# Autodesk Inventor assembly: battery gate
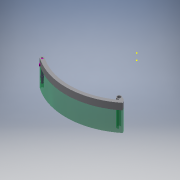
[picture p0: Inventor's stored thumbnail of the model, 180x180]
Saved by Autodesk Inventor 2016 (Build 200138000, 138)
## iProperties
Created: 2015-09-29
Part Number: battery gate
Document SubType Name: Assembly
Designer: Hulbert Office
Author: Hulbert Office
## Documents named in this file (4)
- C:\Users\Hulbert Office\Dropbox\SHF Robotics\battery gate.iam
- C:\Users\Hulbert Office\Dropbox\SHF Robotics\battery gate.ipt
- C:\Users\Hulbert Office\Dropbox\SHF Robotics\battery gate upper.ipt
- C:\Users\Hulbert Office\Dropbox\SHF Robotics\battery gate pin.ipt
## Components (3 placed, 3 different names)
1. battery gate:1 — Mate:1, Mate:2, Mate:3, Mate:4
2. battery gate upper:1 — Mate:1, Mate:2, Mate:3
3. battery gate pin:1 — Mate:4
## Relationships (4: Mate 4)
- Mate:1: battery gate:1 ↔ battery gate upper:1
- Mate:2: battery gate:1 ↔ battery gate upper:1
- Mate:3: battery gate:1 ↔ battery gate upper:1
- Mate:4: battery gate:1 ↔ battery gate pin:1
